# Autodesk Inventor assembly: immersion_chamber
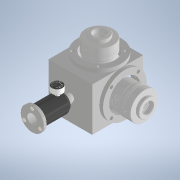
[picture p0: Inventor's stored thumbnail of the model, 180x180]
Saved by Autodesk Inventor 2021 (Build 250183000, 183)
## iProperties
Created: 2021-06-16
Part Number: immersion_chamber
Document SubType Name: Assembly
Designer: MicroscopyInnovation
Author: MicroscopyInnovation
## Documents named in this file (6)
- C:\Users\MicroscopyInnovation\Documents\Inventor\NatProtocolsManuscript\immersion_chamber.iam
- C:\Users\MicroscopyInnovation\Documents\Inventor\NatProtocolsManuscript\immersion_chamber_bath.ipt
- C:\Users\MicroscopyInnovation\Documents\Inventor\NatProtocolsManuscript\immersion_chamber_plate.ipt
- C:\Users\MicroscopyInnovation\Documents\Inventor\NatProtocolsManuscript\TR1-Step.ipt
- C:\Users\MicroscopyInnovation\Documents\Inventor\NatProtocolsManuscript\PH1.5E.ipt
- C:\Users\MicroscopyInnovation\Documents\Inventor\NatProtocolsManuscript\1-26990 (54-10-12 @ 480-910nm) REV C.ipt
## Components (7 placed, 5 different names)
1. immersion_chamber_bath:1 — Mate:1, Mate:2, Mate:3, Mate:4, Mate:5, Mate:6, Mate:7, Mate:8, Mate:9, Mate:11, Mate:12, Mate:13
2. immersion_chamber_plate:1 — Mate:1, Mate:2, Mate:3, Mate:4
3. immersion_chamber_plate:2 — Mate:5, Mate:6, Mate:7
4. TR1-Step:1 — Mate:8, Mate:9, Mate:10
5. PH1.5E:1 — Mate:10, Mate:11
6. 1-26990 (54-10-12 @ 480-910nm) REV C:1 — Mate:12
7. 1-26990 (54-10-12 @ 480-910nm) REV C:2 — Mate:13
## Relationships (13: Mate 13)
- Mate:1: immersion_chamber_bath:1 ↔ immersion_chamber_plate:1
- Mate:2: immersion_chamber_bath:1 ↔ immersion_chamber_plate:1
- Mate:3: immersion_chamber_bath:1 ↔ immersion_chamber_plate:1
- Mate:4: immersion_chamber_bath:1 ↔ immersion_chamber_plate:1
- Mate:5: immersion_chamber_bath:1 ↔ immersion_chamber_plate:2
- Mate:6: immersion_chamber_bath:1 ↔ immersion_chamber_plate:2
- Mate:7: immersion_chamber_bath:1 ↔ immersion_chamber_plate:2
- Mate:8: immersion_chamber_bath:1 ↔ TR1-Step:1
- Mate:9: immersion_chamber_bath:1 ↔ TR1-Step:1
- Mate:10: TR1-Step:1 ↔ PH1.5E:1
- Mate:11 (10 mm): immersion_chamber_bath:1 ↔ PH1.5E:1
- Mate:12: immersion_chamber_bath:1 ↔ 1-26990 (54-10-12 @ 480-910nm) REV C:1
- Mate:13: immersion_chamber_bath:1 ↔ 1-26990 (54-10-12 @ 480-910nm) REV C:2
